# Autodesk Inventor assembly: LEAD NUT ASSEMBLY
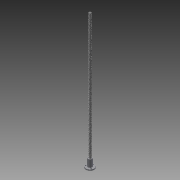
[picture p0: Inventor's stored thumbnail of the model, 180x180]
Saved by Autodesk Inventor 2013 (Build 170138000, 138)
## iProperties
Created: 2013-12-08
Part Number: LEAD NUT ASSEMBLY
Document SubType Name: Assembly
Designer: employee
Author: employee
## Documents named in this file (3)
- C:\Users\employee\Desktop\ConceptFORGE\ConceptFORGE\LISA Simpson\INVENTOR FILES\LEAD NUT ASSEMBLY.iam
- C:\Users\employee\Desktop\ConceptFORGE\ConceptFORGE\LISA Simpson\INVENTOR FILES\_LEAD NUT BLANK.ipt
- C:\Users\employee\Desktop\ConceptFORGE\ConceptFORGE\LISA Simpson\INVENTOR FILES\7_16 TORQSPLINE.ipt
## Components (2 placed, 2 different names)
1. _LEAD NUT BLANK:1 — Mate:1, Flush:1
2. 7_16 TORQSPLINE:1 — Mate:1, Flush:1
## Relationships (2: Mate 1, Flush 1)
- Mate:1: _LEAD NUT BLANK:1 ↔ 7_16 TORQSPLINE:1
- Flush:1: _LEAD NUT BLANK:1 ↔ 7_16 TORQSPLINE:1
